# Autodesk Inventor assembly: Electric-Scooter
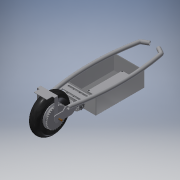
[picture p0: Inventor's stored thumbnail of the model, 180x180]
Saved by Autodesk Inventor 2018 (Build 220112000, 112)
## iProperties
Created: 2018-08-10
Part Number: Electric-Scooter
Document SubType Name: Assembly
Designer: ruben
Author: ruben
## Documents named in this file (7)
- C:\Users\ruben\Documents\Inventor\Electric-Scooter\Electric-Scooter.iam
- C:\Users\ruben\Documents\Inventor\Electric-Scooter\Frame\Frame.iam
- C:\Users\ruben\Documents\Inventor\Electric-Scooter\Transmission\Rear Wheel Axle.ipt
- C:\Users\ruben\Documents\Inventor\Electric-Scooter\Transmission\Real Wheel + Sprocket.iam
- C:\Users\ruben\Documents\Inventor\Electric-Scooter\Transmission\Motor + sprocket + translock.iam
- C:\Users\ruben\Documents\Inventor\Electric-Scooter\Transmission\Motor holder.ipt
- C:\Users\ruben\Documents\Inventor\Electric-Scooter\Transmission\Motor holder slider.ipt
## Components (6 placed, 6 different names)
1. Frame:1 [sub-assembly] — Insert:1, Mate:2, Mate:3, Mate:4
2. Rear Wheel Axle:1 — Insert:1, Insert:2
3. Real Wheel + Sprocket:1 [sub-assembly] — Insert:2, Flush:1
4. Motor + sprocket + translock:1 [sub-assembly] — Flush:1, Insert:3, Insert:4
5. Motor holder:1 — Insert:3, Insert:4, Flush:2, Mate:5
6. Motor holder slider:1 — Mate:2, Mate:3, Mate:4, Flush:2, Mate:5
## Relationships (10: Insert 4, Mate 4, Flush 2)
- Insert:1 (0.5 mm): Frame:1 ↔ Rear Wheel Axle:1
- Insert:2 (8.4 mm): Rear Wheel Axle:1 ↔ Real Wheel + Sprocket:1
- Flush:1: Real Wheel + Sprocket:1 ↔ Motor + sprocket + translock:1
- Insert:3: Motor + sprocket + translock:1 ↔ Motor holder:1
- Insert:4: Motor + sprocket + translock:1 ↔ Motor holder:1
- Mate:2: Frame:1 ↔ Motor holder slider:1
- Mate:3: Frame:1 ↔ Motor holder slider:1
- Mate:4: Frame:1 ↔ Motor holder slider:1
- Flush:2: Motor holder:1 ↔ Motor holder slider:1
- Mate:5: Motor holder:1 ↔ Motor holder slider:1
